# Autodesk Inventor assembly: SimpleBase_Segment
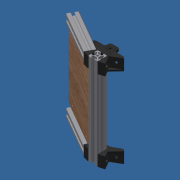
[picture p0: Inventor's stored thumbnail of the model, 180x180]
Saved by Autodesk Inventor 2014 SP2 (Build 180246200, 246)
## iProperties
Created: 2015-02-08
Part Number: SimpleBase_Segment
Document SubType Name: Assembly
Designer: 4ndreas
Author: 4ndreas
## Documents named in this file (5)
- C:\Users\4ndreas\Documents\Inventor\RobotARM v2\Base\SimpleBase_Segment.iam
- C:\Users\4ndreas\Documents\Inventor\RobotARM v2\Base\Strebe_hex_1x.ipt
- C:\Users\4ndreas\Documents\Inventor\Pentagon 3D printer\Hexagon\hexagon_top_v_2_0_x1.ipt
- C:\Users\4ndreas\Documents\Inventor\RobotARM v2\Base\Strebe_hoehe_hex_1x.ipt
- C:\Users\4ndreas\Documents\Inventor\RobotARM v2\Base\SeitenWand.ipt
## Components (6 placed, 4 different names)
1. SeitenWand:1 — Passend:45, Passend:46, Passend:47
2. hexagon_top_v_2_0_x1:3 — Fluchtend:23, Passend:23, Passend:24, Passend:25, Passend:26, Passend:44, Passend:46, Passend:47, Passend:49, Passend:50
3. Strebe_hex_1x:5 — Passend:23, Passend:26, Passend:44, Passend:45
4. Strebe_hoehe_hex_1x:4 — Fluchtend:20, Passend:20, Passend:21, Fluchtend:23, Passend:24, Passend:25, Passend:48
5. hexagon_top_v_2_0_x1:2 — Passend:13, Passend:14, Fluchtend:16, Fluchtend:20, Passend:20, Passend:21
6. Strebe_hex_1x:2 — Passend:13, Passend:14, Fluchtend:16
## Relationships (18: Mate 15, Flush 3)
- Passend:13 [Mate]: hexagon_top_v_2_0_x1:2 ↔ Strebe_hex_1x:2
- Passend:14 [Mate]: hexagon_top_v_2_0_x1:2 ↔ Strebe_hex_1x:2
- Fluchtend:16 [Flush]: hexagon_top_v_2_0_x1:2 ↔ Strebe_hex_1x:2
- Fluchtend:20 [Flush]: Strebe_hoehe_hex_1x:4 ↔ hexagon_top_v_2_0_x1:2
- Passend:20 [Mate]: Strebe_hoehe_hex_1x:4 ↔ hexagon_top_v_2_0_x1:2
- Passend:21 [Mate]: Strebe_hoehe_hex_1x:4 ↔ hexagon_top_v_2_0_x1:2
- Fluchtend:23 [Flush]: hexagon_top_v_2_0_x1:3 ↔ Strebe_hoehe_hex_1x:4
- Passend:23 [Mate]: hexagon_top_v_2_0_x1:3 ↔ Strebe_hex_1x:5
- Passend:24 [Mate]: hexagon_top_v_2_0_x1:3 ↔ Strebe_hoehe_hex_1x:4
- Passend:25 [Mate]: hexagon_top_v_2_0_x1:3 ↔ Strebe_hoehe_hex_1x:4
- Passend:26 [Mate]: hexagon_top_v_2_0_x1:3 ↔ Strebe_hex_1x:5
- Passend:44 [Mate]: hexagon_top_v_2_0_x1:3 ↔ Strebe_hex_1x:5
- Passend:45 [Mate]: SeitenWand:1 ↔ Strebe_hex_1x:5
- Passend:46 [Mate]: SeitenWand:1 ↔ hexagon_top_v_2_0_x1:3
- Passend:47 [Mate]: SeitenWand:1 ↔ hexagon_top_v_2_0_x1:3
- Passend:49 [Mate]: hexagon_top_v_2_0_x1:3
- Passend:48 [Mate]: Strebe_hoehe_hex_1x:4
- Passend:50 [Mate]: hexagon_top_v_2_0_x1:3
